# Autodesk Inventor assembly: head_assembly
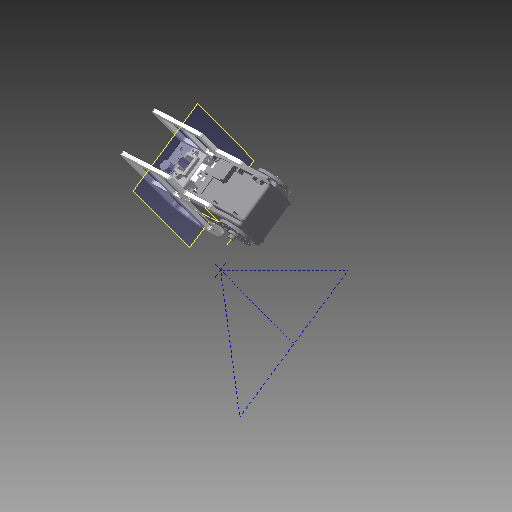
[picture p0: Inventor's stored thumbnail of the model, 512x512]
Saved by Autodesk Inventor 2018 (Build 220112000, 112)
## iProperties
Created: 2018-04-23
Part Number: head_assembly
Document SubType Name: Assembly
Designer: medrimonia
Author: medrimonia
## Documents named in this file (6)
- C:\Users\etd\Dropbox\SigmaBan\SigmaBanV2.1\head_mx64\head_assembly.iam
- C:\Users\etd\Dropbox\SigmaBan\SigmaBanV2.1\head_mx64\ptgrey_fix2.ipt
- C:\Users\etd\Dropbox\SigmaBan\SigmaBanV2.1\head_mx64\base_head.ipt
- C:\Users\etd\Dropbox\SigmaBan\SigmaBanV2.1\PtGreyCamera_full.ipt
- C:\Users\etd\Dropbox\SigmaBan\SigmaBanV2.1\MX-64AT_AR_contreaxe.iam
- C:\Users\etd\Dropbox\SigmaBan\SigmaBanV2.1\obj.ipt
## Components (6 placed, 5 different names)
1. ptgrey_fix2:1 — Mate:1, Mate:3, Mate:4, Mate:6, Mate:7, Mate:8, Mate:9, Mate:17
2. base_head:1 — Mate:1, Mate:3, Mate:11, Mate:12, Mate:16
3. base_head:2 — Mate:4, Mate:6, Mate:10, Mate:17
4. PtGreyCamera_full:1 — Mate:7, Mate:8, Mate:9, Mate:13, Mate:14, Mate:15, Angle:1
5. Motor:head_pitch [sub-assembly] — Mate:10, Mate:11, Mate:12, Mate:16
6. obj:1 — Mate:13, Mate:14
## Relationships (16: Mate 15, Angle 1)
- Mate:1: ptgrey_fix2:1 ↔ base_head:1
- Mate:3: ptgrey_fix2:1 ↔ base_head:1
- Mate:4: ptgrey_fix2:1 ↔ base_head:2
- Mate:6: ptgrey_fix2:1 ↔ base_head:2
- Mate:7: ptgrey_fix2:1 ↔ PtGreyCamera_full:1
- Mate:8: ptgrey_fix2:1 ↔ PtGreyCamera_full:1
- Mate:9: ptgrey_fix2:1 ↔ PtGreyCamera_full:1
- Mate:10: base_head:2 ↔ Motor:head_pitch
- Mate:11: base_head:1 ↔ Motor:head_pitch
- Mate:12: base_head:1 ↔ Motor:head_pitch
- Mate:13: PtGreyCamera_full:1 ↔ obj:1
- Mate:14: PtGreyCamera_full:1 ↔ obj:1
- Mate:15: PtGreyCamera_full:1
- Angle:1 (0 deg): PtGreyCamera_full:1
- Mate:16: base_head:1 ↔ Motor:head_pitch
- Mate:17: ptgrey_fix2:1 ↔ base_head:2
## Named parameters: viewAngle = 65 deg
